# Autodesk Inventor assembly: Estante Dofbot
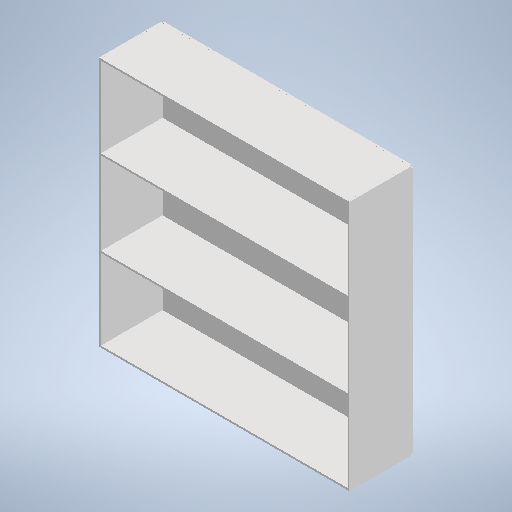
[picture p0: Inventor's stored thumbnail of the model, 512x512]
Saved by Autodesk Inventor 2025.1 (Build 291241020, 241B)
## iProperties
Created: 2024-11-13
Part Number: Estante Dofbot
Document SubType Name: Assembly
Designer: marco
Author: marco
## Documents named in this file (5)
- C:\Users\marco\Downloads\Estante Dofbot.iam
- C:\Users\marco\Downloads\Lateral sup e inf.ipt
- C:\Users\marco\Downloads\Base sup e inf.ipt
- C:\Users\marco\Downloads\Pared estanteria.ipt
- C:\Users\marco\Downloads\Estante int.ipt
## Components (7 placed, 4 different names)
1. Lateral sup e inf:1 — Mate:1, Mate:2, Mate:3, Mate:11
2. Base sup e inf:1 — Mate:3, Mate:4, Mate:5, Mate:6, Mate:7, Mate:8, Mate:9, Mate:10
3. Pared estanteria:1 — Mate:1, Mate:2, Mate:4, Mate:12
4. Estante int:1 — Mate:5, Mate:6
5. Estante int:2 — Mate:7, Mate:8
6. Base sup e inf:2 — Mate:11, Mate:12
7. Lateral sup e inf:2 — Mate:9, Mate:10
## Relationships (12: Mate 12)
- Mate:1: Lateral sup e inf:1 ↔ Pared estanteria:1
- Mate:2: Lateral sup e inf:1 ↔ Pared estanteria:1
- Mate:3: Lateral sup e inf:1 ↔ Base sup e inf:1
- Mate:4: Base sup e inf:1 ↔ Pared estanteria:1
- Mate:5: Base sup e inf:1 ↔ Estante int:1
- Mate:6: Base sup e inf:1 ↔ Estante int:1
- Mate:7: Base sup e inf:1 ↔ Estante int:2
- Mate:8: Base sup e inf:1 ↔ Estante int:2
- Mate:9: Base sup e inf:1 ↔ Lateral sup e inf:2
- Mate:10: Base sup e inf:1 ↔ Lateral sup e inf:2
- Mate:11: Lateral sup e inf:1 ↔ Base sup e inf:2
- Mate:12: Pared estanteria:1 ↔ Base sup e inf:2
